# Autodesk Inventor assembly: mg996r_rot_into_rot
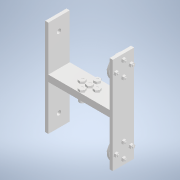
[picture p0: Inventor's stored thumbnail of the model, 180x180]
Saved by Autodesk Inventor 2021.4 (Build 254397000, 397)
## iProperties
Created: 2022-07-24
Part Number: mg996r_rot_into_rot
Document SubType Name: Assembly
Designer: isamu
Author: isamu
## Documents named in this file (4)
- D:\personal_projects\robot\inventor\2021_export_exp\mg996r_rot_into_rot.iam
- D:\personal_projects\robot\inventor\2021_export_exp\mg996r_rot_frame.iam
- D:\personal_projects\robot\exports\screws\m3x8.ipt
- D:\personal_projects\robot\exports\screws\m3 nuts.ipt
## Components (12 placed, 3 different names)
1. mg996r_rot_frame:1 [sub-assembly] — Mate:1, Mate:2, Mate:3, Insert:1, Insert:2, Insert:3, Insert:4, Insert:5
2. mg996r_rot_frame:2 [sub-assembly] — Mate:1, Mate:2, Mate:3, Insert:6, Insert:7, Insert:8, Insert:9, Insert:10
3. m3x8:1 — Insert:2
4. m3x8:2 — Insert:4
5. m3x8:3 — Insert:3
6. m3x8:4 — Insert:5
7. m3x8:5 — Insert:1
8. m3 nuts:1 — Insert:6
9. m3 nuts:2 — Insert:7
10. m3 nuts:3 — Insert:8
11. m3 nuts:4 — Insert:10
12. m3 nuts:5 — Insert:9
## Relationships (13: Insert 10, Mate 3)
- Mate:1: mg996r_rot_frame:1 ↔ mg996r_rot_frame:2
- Mate:2: mg996r_rot_frame:1 ↔ mg996r_rot_frame:2
- Mate:3: mg996r_rot_frame:1 ↔ mg996r_rot_frame:2
- Insert:1: mg996r_rot_frame:1 ↔ m3x8:5
- Insert:2: mg996r_rot_frame:1 ↔ m3x8:1
- Insert:3: mg996r_rot_frame:1 ↔ m3x8:3
- Insert:4: mg996r_rot_frame:1 ↔ m3x8:2
- Insert:5: mg996r_rot_frame:1 ↔ m3x8:4
- Insert:6: mg996r_rot_frame:2 ↔ m3 nuts:1
- Insert:7: mg996r_rot_frame:2 ↔ m3 nuts:2
- Insert:8: mg996r_rot_frame:2 ↔ m3 nuts:3
- Insert:9: mg996r_rot_frame:2 ↔ m3 nuts:5
- Insert:10: mg996r_rot_frame:2 ↔ m3 nuts:4
